# Autodesk Inventor assembly: złożeniówka1
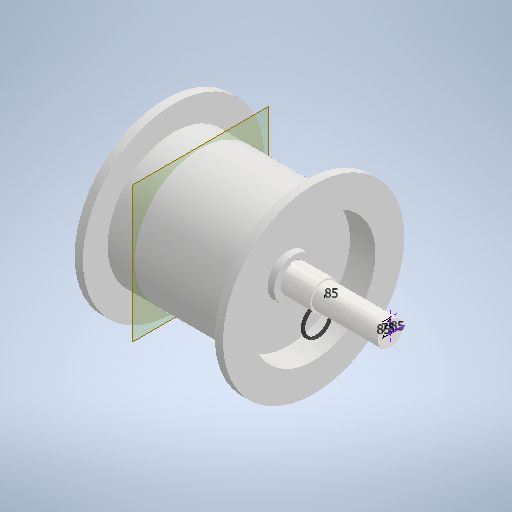
[picture p0: Inventor's stored thumbnail of the model, 512x512]
Saved by Autodesk Inventor 2025 (Build 290162000, 162)
## iProperties
Created: 2025-05-18
Part Number: złożeniówka1
Document SubType Name: Assembly
Designer: PC
Author: PC
## Documents named in this file (7)
- C:\Users\PC\Desktop\złożeniówka1.iam
- C:\Users\PC\Desktop\Wał4.ipt
- C:\Users\PC\Documents\Inventor\Content Center Files\R2025\pl-PL\BS 290 SKF(05)\BS 290 SKF - SKF QJ 230 N2.ipt
- C:\Users\PC\Documents\Inventor\Content Center Files\R2025\pl-PL\DIN 3760 A\DIN 3760 - A - 150 x 180 x 15 - NBR.ipt
- C:\Users\PC\Downloads\1415151513515.ipt
- C:\Users\PC\Desktop\wał naszz\Design Accelerator\Połączenie wpustowe3.iam
- C:\Users\PC\Desktop\wał naszz\Design Accelerator\Połączenie wpustowe4.iam
## Components (7 placed, 5 different names)
1. Wał:1 — Obrotowe:1, Obrotowe:2, Równoległe:1, Zestawiające:4, Równoległe:3, Kątowe:1, Zestawiające:5, Równoległe:4, Kątowe:2, Zestawiające:6, Kątowe:3
2. BS 290 SKF- do styku czteropunktowego SKF QJ 230 N2:1 — Obrotowe:2, Zestawiające:1, Zestawiające:2, Zestawiające:3
3. BS 290 SKF- do styku czteropunktowego SKF QJ 230 N2:2 — Obrotowe:1
4. DIN 3760 A A - 150 x 180 x 15 - NBR:1
5. 1415151513515:1 — Zestawiające:4, Kątowe:3
6. Połączenie wpustowe:1 [sub-assembly] — Równoległe:3, Kątowe:1, Zestawiające:5
7. Połączenie wpustowe:2 [sub-assembly] — Równoległe:4, Kątowe:2, Zestawiające:6
## Relationships (15: Mate 6, Flush 4, Angle 3, RevoluteJoint 2)
- Obrotowe:1 [RevoluteJoint] (358 mm): Wał:1 ↔ BS 290 SKF- do styku czteropunktowego SKF QJ 230 N2:2
- Obrotowe:2 [RevoluteJoint] (-156 mm): Wał:1 ↔ BS 290 SKF- do styku czteropunktowego SKF QJ 230 N2:1
- Równoległe:1 [Flush]: Wał:1
- Zestawiające:1 [Mate]: BS 290 SKF- do styku czteropunktowego SKF QJ 230 N2:1
- Zestawiające:2 [Mate]: BS 290 SKF- do styku czteropunktowego SKF QJ 230 N2:1
- Zestawiające:3 [Mate]: BS 290 SKF- do styku czteropunktowego SKF QJ 230 N2:1
- Równoległe:2 [Flush] (-200 mm)
- Zestawiające:4 [Mate] (180 mm): Wał:1 ↔ 1415151513515:1
- Równoległe:3 [Flush] (205.0064 mm): Wał:1 ↔ Połączenie wpustowe:1
- Kątowe:1 [Angle] (180 deg): Wał:1 ↔ Połączenie wpustowe:1
- Zestawiające:5 [Mate]: Wał:1 ↔ Połączenie wpustowe:1
- Równoległe:4 [Flush] (204.9978 mm): Wał:1 ↔ Połączenie wpustowe:2
- Kątowe:2 [Angle] (0 deg): Wał:1 ↔ Połączenie wpustowe:2
- Zestawiające:6 [Mate]: Wał:1 ↔ Połączenie wpustowe:2
- Kątowe:3 [Angle] (90 deg): Wał:1 ↔ 1415151513515:1
